# Autodesk Inventor assembly: Nixie Tester
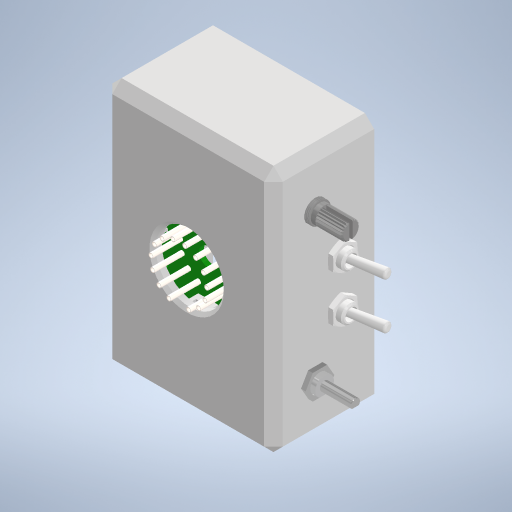
[picture p0: Inventor's stored thumbnail of the model, 512x512]
Saved by Autodesk Inventor 2024 (Build 280153000, 153)
## iProperties
Created: 2025-09-18
Part Number: Nixie Tester
Document SubType Name: Assembly
Designer: Login
Author: Login
## Documents named in this file (7)
- D:\Inventor\Repositories\Nixie-Tester\Nixie Tester.iam
- D:\Inventor\Repositories\Nixie-Tester\Import\Altium\Nixie Tester_Step_Rev.1.0._2025-09-18\Nixie Tester_Step_Rev.1.0._2025-09-18.ipt
- D:\Inventor\Repositories\Nixie-Tester\Nixie Tester TOP.ipt
- D:\Inventor\Repositories\Common\Components\6mm DPDT Mini Toggle Switch.iam
- D:\Inventor\Repositories\Common\Components\6mm SPDT Mini Toggle Switch.iam
- D:\Inventor\Repositories\Common\Components\Rotory Switch 6mm 10 pole.ipt
- D:\Inventor\Repositories\Common\Components\Mono potmeter.ipt
## Components (6 placed, 6 different names)
1. Nixie Tester_Step_Rev.1.0._2025-09-18:1 — Insert:1, Insert:2, Insert:3, Insert:4
2. Nixie Tester TOP:1 — Insert:1, Insert:2, Insert:3, Insert:4, Mate:1, Mate:2, Insert:7, Angle:3, Insert:9, Insert:10, Angle:4, Angle:5, Angle:6, Insert:11
3. 6mm DPDT Mini Toggle Switch:1 [sub-assembly] — Insert:10, Angle:5
4. 6mm SPDT Mini Toggle Switch:1 [sub-assembly] — Insert:9, Angle:4
5. Rotory Switch 6mm 10 pole:1 — Insert:7, Angle:3
6. Mono potmeter:1 — Angle:6, Insert:11
## Relationships (14: Insert 8, Angle 4, Mate 2)
- Insert:1: Nixie Tester_Step_Rev.1.0._2025-09-18:1 ↔ Nixie Tester TOP:1
- Insert:2: Nixie Tester_Step_Rev.1.0._2025-09-18:1 ↔ Nixie Tester TOP:1
- Insert:3: Nixie Tester_Step_Rev.1.0._2025-09-18:1 ↔ Nixie Tester TOP:1
- Insert:4: Nixie Tester_Step_Rev.1.0._2025-09-18:1 ↔ Nixie Tester TOP:1
- Mate:1: Nixie Tester TOP:1
- Mate:2: Nixie Tester TOP:1
- Insert:7: Nixie Tester TOP:1 ↔ Rotory Switch 6mm 10 pole:1
- Angle:3 (0 deg): Nixie Tester TOP:1 ↔ Rotory Switch 6mm 10 pole:1
- Insert:9: Nixie Tester TOP:1 ↔ 6mm SPDT Mini Toggle Switch:1
- Insert:10: Nixie Tester TOP:1 ↔ 6mm DPDT Mini Toggle Switch:1
- Angle:4 (0 deg): Nixie Tester TOP:1 ↔ 6mm SPDT Mini Toggle Switch:1
- Angle:5 (0 deg): Nixie Tester TOP:1 ↔ 6mm DPDT Mini Toggle Switch:1
- Angle:6 (0 deg): Nixie Tester TOP:1 ↔ Mono potmeter:1
- Insert:11: Nixie Tester TOP:1 ↔ Mono potmeter:1
